# Autodesk Inventor assembly: Cruz de malta
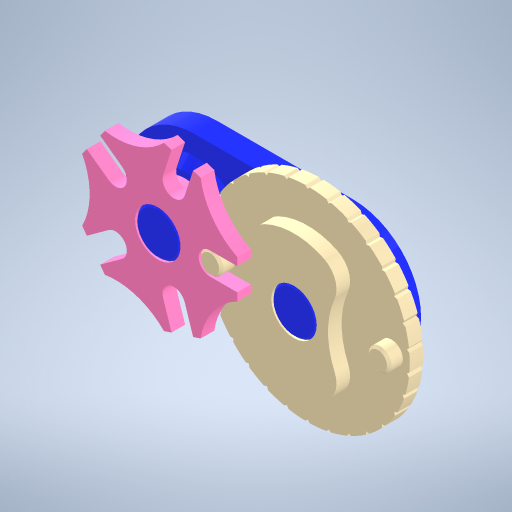
[picture p0: Inventor's stored thumbnail of the model, 512x512]
Saved by Autodesk Inventor 2023 (Build 270158000, 158)
## iProperties
Created: 2023-03-20
Part Number: Cruz de malta
Document SubType Name: Assembly
Designer: jpjoa
Author: jpjoa
## Documents named in this file (4)
- G:\.shortcut-targets-by-id\1lOMf-Kp8UroJbDMtxyO7ak_I_KYCWiat\Faculdade\in class\Inventor\04\Cruz de malta.iam
- G:\.shortcut-targets-by-id\1lOMf-Kp8UroJbDMtxyO7ak_I_KYCWiat\Faculdade\in class\Inventor\03\Conjunto\base.ipt
- G:\.shortcut-targets-by-id\1lOMf-Kp8UroJbDMtxyO7ak_I_KYCWiat\Faculdade\in class\Inventor\03\Conjunto\cruz de malta.ipt
- G:\.shortcut-targets-by-id\1lOMf-Kp8UroJbDMtxyO7ak_I_KYCWiat\Faculdade\in class\Inventor\03\Conjunto\manivela.ipt
## Components (3 placed, 3 different names)
1. base:1 — Mate:1, Mate:2, Insert:1, Angle:1
2. cruz de malta:1 — Mate:1, Mate:2
3. manivela:1 — Insert:1, Angle:1
## Relationships (4: Mate 2, Insert 1, Angle 1)
- Mate:1: base:1 ↔ cruz de malta:1
- Mate:2: base:1 ↔ cruz de malta:1
- Insert:1: base:1 ↔ manivela:1
- Angle:1 (0 deg): base:1 ↔ manivela:1
